# Autodesk Inventor assembly: main
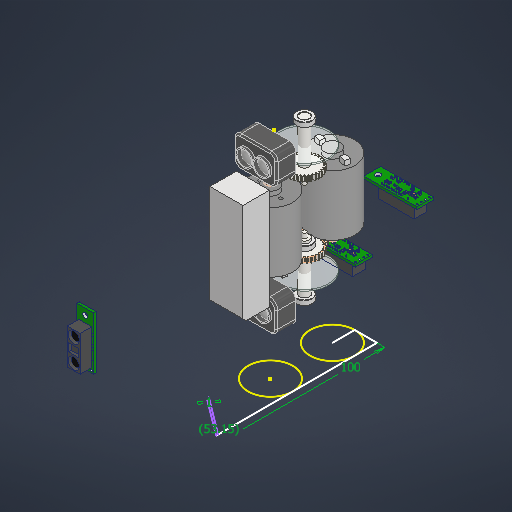
[picture p0: Inventor's stored thumbnail of the model, 512x512]
Saved by Autodesk Inventor 2026.2 (Build 302298000, 298)
## iProperties
Created: 2026-03-09
Part Number: main
Document SubType Name: Assembly
Designer: szymo
Author: szymo
## Documents named in this file (9)
- C:\Users\szymo\Downloads\evangelion-turbo\inventor-project\main.iam
- C:\Users\szymo\Downloads\evangelion-turbo\inventor-project\drive-train.iam
- C:\Users\szymo\Downloads\evangelion-turbo\inventor-project\LUNA.ipt
- C:\Users\szymo\Downloads\evangelion-turbo\inventor-project\2s450mahSHORT.ipt
- C:\Users\szymo\Downloads\evangelion-turbo\inventor-project\2s450mah.ipt
- C:\Users\szymo\Downloads\evangelion-turbo\inventor-project\3s550mah.ipt
- C:\Users\szymo\Downloads\evangelion-turbo\inventor-project\2s550mah.ipt
- C:\Users\szymo\Downloads\evangelion-turbo\inventor-project\3s450mah.ipt
- C:\Users\szymo\Downloads\evangelion-turbo\inventor-project\sharp\sharp\sharp.ipt
## Components (11 placed, 8 different names)
1. drive-train:1 [sub-assembly]
2. LUNA:2
3. LUNA:1
4. sharp:1
5. sharp:2
6. sharp:3
7. 2s450mahSHORT:1
8. 2s450mah:1
9. 3s550mah:1
10. 2s550mah:1
11. 3s450mah:1
## Relationships (1: Flush 1)
- Flush:1 (-101.75 mm)
